# Autodesk Inventor assembly: Frame
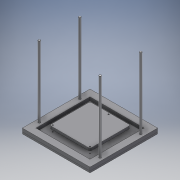
[picture p0: Inventor's stored thumbnail of the model, 180x180]
Saved by Autodesk Inventor 2016 (Build 200138000, 138)
## iProperties
Created: 2017-05-15
Part Number: Frame
Document SubType Name: Assembly
Designer: 31745
Author: 31745
## Documents named in this file (6)
- H:\Projects\Printer #2\Printer2\IAM\Frame.iam
- H:\Projects\Printer #2\Printer2\IPT\Machined Parts\Base.ipt
- H:\Projects\Printer #2\Printer2\IPT\Machined Parts\Print Bed.ipt
- H:\Projects\Printer #2\Printer2\IPT\Machined Parts\XY Carriage.ipt
- H:\Projects\Printer #2\Printer2\IPT\Machined Parts\Smooth Rod Brace Bottom.ipt
- H:\Projects\Printer #2\Printer2\IPT\Purchased Parts\8mm smooth rod.ipt
## Components (8 placed, 5 different names)
1. Base:1 — Mate:1, Mate:2, Flush:1, Flush:2, Mate:3, Mate:4, Flush:3, Flush:4, Mate:9, Mate:10, Mate:11, Mate:12
2. Print Bed:1 — Mate:1, Mate:2, Mate:3
3. XY Carriage:1 — Flush:1, Flush:2
4. Smooth Rod Brace Bottom:1 — Mate:4, Flush:3, Flush:4, Mate:5, Mate:6, Mate:7, Mate:8
5. 8mm smooth rod:1 — Mate:8, Mate:11
6. 8mm smooth rod:2 — Mate:5, Mate:9
7. 8mm smooth rod:3 — Mate:7, Mate:10
8. 8mm smooth rod:4 — Mate:6, Mate:12
## Relationships (16: Mate 12, Flush 4)
- Mate:1: Base:1 ↔ Print Bed:1
- Mate:2: Base:1 ↔ Print Bed:1
- Flush:1: Base:1 ↔ XY Carriage:1
- Flush:2: Base:1 ↔ XY Carriage:1
- Mate:3 (12.7 mm): Base:1 ↔ Print Bed:1
- Mate:4: Base:1 ↔ Smooth Rod Brace Bottom:1
- Flush:3: Base:1 ↔ Smooth Rod Brace Bottom:1
- Flush:4: Base:1 ↔ Smooth Rod Brace Bottom:1
- Mate:5: Smooth Rod Brace Bottom:1 ↔ 8mm smooth rod:2
- Mate:6: Smooth Rod Brace Bottom:1 ↔ 8mm smooth rod:4
- Mate:7: Smooth Rod Brace Bottom:1 ↔ 8mm smooth rod:3
- Mate:8: Smooth Rod Brace Bottom:1 ↔ 8mm smooth rod:1
- Mate:9: Base:1 ↔ 8mm smooth rod:2
- Mate:10: Base:1 ↔ 8mm smooth rod:3
- Mate:11: Base:1 ↔ 8mm smooth rod:1
- Mate:12: Base:1 ↔ 8mm smooth rod:4
